# Autodesk Inventor assembly: Zusammenbau
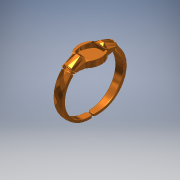
[picture p0: Inventor's stored thumbnail of the model, 180x180]
Saved by Autodesk Inventor 2019 (Build 230136000, 136)
## iProperties
Created: 2021-03-09
Part Number: Zusammenbau
Material: Generisch
Document SubType Name: Assembly
Designer: Bergi
Author: Bergi
## Documents named in this file (5)
- C:\Users\Bergi\Desktop\3D Sketches\Bulova\Zusammenbau.iam
- C:\Users\Bergi\Desktop\3D Sketches\Bulova\Main_afterRhino.ipt
- C:\Users\Bergi\Desktop\3D Sketches\Bulova\bild.ipt
- C:\Users\Bergi\Desktop\3D Sketches\Bulova\Armband_afterrhino.ipt
- C:\Users\Bergi\Desktop\3D Sketches\Bulova\Deckel.ipt
## Components (5 placed, 4 different names)
1. Main_afterRhino:1 — Passend:1, Passend:2, Fluchtend:1, Fluchtend:2, Passend:3, Passend:4
2. bild:1
3. Armband_afterrhino:1 — Passend:1, Fluchtend:1
4. Armband_afterrhino:2 — Passend:2, Fluchtend:2
5. Deckel:1 — Passend:3, Passend:4
## Relationships (6: Mate 4, Flush 2)
- Passend:1 [Mate]: Main_afterRhino:1 ↔ Armband_afterrhino:1
- Passend:2 [Mate]: Main_afterRhino:1 ↔ Armband_afterrhino:2
- Fluchtend:1 [Flush]: Main_afterRhino:1 ↔ Armband_afterrhino:1
- Fluchtend:2 [Flush]: Main_afterRhino:1 ↔ Armband_afterrhino:2
- Passend:3 [Mate]: Main_afterRhino:1 ↔ Deckel:1
- Passend:4 [Mate]: Main_afterRhino:1 ↔ Deckel:1
